# Autodesk Inventor assembly: door_wo_glass
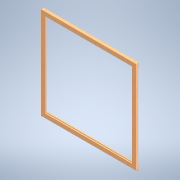
[picture p0: Inventor's stored thumbnail of the model, 180x180]
Saved by Autodesk Inventor 2020 (Build 240168000, 168)
## iProperties
Created: 2020-05-19
Part Number: door_wo_glass
Document SubType Name: Assembly
Designer: kolbe
Author: kolbe
## Documents named in this file (4)
- C:\Users\kolbe\Documents\GitHub\Terrarium\door\door_wo_glass.iam
- C:\Users\kolbe\Documents\GitHub\Terrarium\door\bottomv2.ipt
- C:\Users\kolbe\Documents\GitHub\Terrarium\door\sidev2.ipt
- C:\Users\kolbe\Documents\GitHub\Terrarium\door\topv2.ipt
## Components (4 placed, 3 different names)
1. bottomv2:1 — Mate:1, Mate:2, Mate:3, Mate:4
2. sidev2:1 — Mate:1, Mate:2, Mate:5, Mate:6
3. sidev2:2 — Mate:3, Mate:4
4. topv2:2 — Mate:5, Mate:6
## Relationships (6: Mate 6)
- Mate:1: bottomv2:1 ↔ sidev2:1
- Mate:2: bottomv2:1 ↔ sidev2:1
- Mate:3: bottomv2:1 ↔ sidev2:2
- Mate:4: bottomv2:1 ↔ sidev2:2
- Mate:5: sidev2:1 ↔ topv2:2
- Mate:6: sidev2:1 ↔ topv2:2
